# Autodesk Inventor assembly: Display.brd
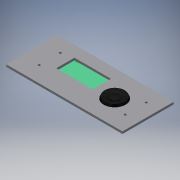
[picture p0: Inventor's stored thumbnail of the model, 180x180]
Saved by Autodesk Inventor 2017.3 (Build 213256000, 256)
## iProperties
Part Number: Display.brd
Material: Generisch
Document SubType Name: Assembly
Designer: Nils
Author: Nils
## Documents named in this file (14)
- C:\Users\Nils\Documents\GitHub\Eurobot2018\Hardware\Display\3D\Display.brd.iam
- C:\Users\Nils\Documents\GitHub\Eurobot2018\Hardware\Display\3D\Display.brd_Kontur.ipt
- C:\Users\Nils\Documents\GitHub\Eurobot2018\Hardware\Display\3D\C0805K, C0805K_1.ipt
- C:\Users\Nils\Documents\GitHub\Eurobot2018\Hardware\Display\3D\ML6, ML6_17.ipt
- C:\Users\Nils\Documents\GitHub\Eurobot2018\Hardware\Display\3D\TQFP32-08, MEGA8-AI_19.ipt
- C:\Users\Nils\Documents\GitHub\Eurobot2018\Hardware\Display\3D\SOT223, REG1117_21.ipt
- C:\Users\Nils\Documents\GitHub\Eurobot2018\Hardware\Display\3D\SOT23, 2N7002_26.ipt
- C:\Users\Nils\Documents\GitHub\Eurobot2018\Hardware\Display\3D\HC49UP, Q3_HC49UP_29.ipt
- C:\Users\Nils\Documents\GitHub\Eurobot2018\Hardware\Display\3D\R0805, R0805_32.ipt
- C:\Users\Nils\Documents\GitHub\Eurobot2018\Hardware\Display\3D\0207_10, 0207_10_37.ipt
- C:\Users\Nils\Documents\GitHub\Eurobot2018\Hardware\Display\3D\LCD-128X64BK_AG, LCD-128X64BK_AG_48.ipt
- C:\Users\Nils\Documents\GitHub\Eurobot2018\Hardware\Display\3D\70597241-9-module_5gth935_1z09136118_4x5eth935\module_5gth935_1z09136118_4x5eth935.iam
- C:\Users\Nils\Documents\GitHub\Eurobot2018\Hardware\Display\3D\Ausschnitt.ipt
- C:\Users\Nils\Documents\GitHub\Eurobot2018\Hardware\Display\3D\LCD-Halterung.ipt
## Components (31 placed, 31 different names)
1. Display.brd_Kontur:1 — Passend:1, Fluchtend:1, Fluchtend:2, Fluchtend:5
2. C1_2
3. C2_3
4. C3_4
5. C4_5
6. C5_6
7. C6_7
8. C7_8
9. C8_9
10. C9_10
11. C10_11
12. C11_12
13. C13_14
14. I2C_18
15. IC1_20
16. IC2_22
17. ISP_23
18. Q1_27
19. Q2_28
20. Q3_30
21. Q4_31
22. R1_33
23. R2_34
24. R3_35
25. R4_36
26. R5_38
27. R6_39
28. U_1_49 — Fluchtend:3
29. module_5gth935_1z09136118_4x5eth935:1 [sub-assembly] — Passend:1, Fluchtend:1, Fluchtend:2
30. Ausschnitt:1 — Fluchtend:3, Fluchtend:4
31. LCD-Halterung:1 — Fluchtend:4, Fluchtend:5
## Relationships (6: Flush 5, Mate 1)
- Passend:1 [Mate]: Display.brd_Kontur:1 ↔ module_5gth935_1z09136118_4x5eth935:1
- Fluchtend:1 [Flush] (19.03 mm): Display.brd_Kontur:1 ↔ module_5gth935_1z09136118_4x5eth935:1
- Fluchtend:2 [Flush] (19.05 mm): Display.brd_Kontur:1 ↔ module_5gth935_1z09136118_4x5eth935:1
- Fluchtend:3 [Flush]: U_1_49 ↔ Ausschnitt:1
- Fluchtend:4 [Flush]: Ausschnitt:1 ↔ LCD-Halterung:1
- Fluchtend:5 [Flush]: Display.brd_Kontur:1 ↔ LCD-Halterung:1
